# Autodesk Inventor assembly: X_Carriage_V2_1
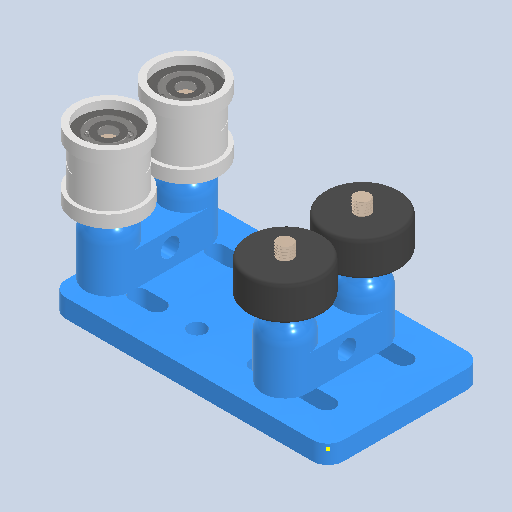
[picture p0: Inventor's stored thumbnail of the model, 512x512]
Saved by Autodesk Inventor 2022 (Build 260153000, 153)
## iProperties
Created: 2021-06-13
Part Number: X_Carriage_V2_1
Document SubType Name: Assembly
Designer: Jorian Brusind
Author: Jorian Brusind
## Documents named in this file (8)
- C:\Users\Jorian Brusind\Documents\GitHub\HyperRail\Inventor Files\X_Carriage_V2_1.iam
- C:\Users\Jorian Brusind\Documents\GitHub\HyperRail\Inventor Files\X_Carriage_Plate.ipt
- C:\Users\Jorian Brusind\Documents\GitHub\HyperRail\Inventor Files\11mm_BearingWheel.ipt
- C:\Users\Jorian Brusind\Documents\GitHub\HyperRail\Inventor Files\4mm_Roller_Spacer_extended.ipt
- C:\Users\Jorian Brusind\Documents\GitHub\HyperRail\Inventor Files\miniature-ball-bearings-metric-series-flanged-1.snapshot.1\F606ZZFlanged\F608 - 8 x 22 x 7.ipt
- C:\Users\Jorian Brusind\Documents\GitHub\PersonalProjects\HyperRail\Inventor Files\miniature-ball-bearings-metric-series-flanged-1.snapshot.1\F606ZZFlanged.ipt
- C:\Users\Jorian Brusind\Documents\GitHub\HyperRail\Inventor Files\685ZZFlanged_Adapter.ipt
- C:\Users\Jorian Brusind\Documents\GitHub\HyperRail\Inventor Files\Metric bolt\Bolt M5 45mm.ipt
## Components (17 placed, 6 different names)
1. X_Carriage_Plate:1 — Mate:51, Mate:53, Mate:65, Angle:1, Mate:66, Angle:2, Mate:98
2. 11mm_BearingWheel:1 — Flush:2, Mate:56, Mate:67
3. 11mm_BearingWheel:4 — Flush:2, Mate:57
4. 4mm_Roller_Spacer_extended:1 — Mate:53, Mate:56, Mate:57, Mate:66, Angle:2, Mate:67, Mate:96, Mate:97
5. 4mm_Roller_Spacer_extended:2 — Mate:51, Mate:65, Angle:1, Mate:76, Mate:77, Mate:78, Mate:79, Mate:94, Mate:95
6. F608 - 8 x 22 x 7:1 — Mate:78, Mate:89, Mate:91
7. F608 - 8 x 22 x 7:2 — Mate:76, Mate:90, Mate:92
8. F608 - 8 x 22 x 7:3 — Mate:79, Mate:84, Mate:85
9. F608 - 8 x 22 x 7:4 — Mate:77, Mate:86, Mate:87
10. 685ZZFlanged_Adapter:1 — Mate:86, Mate:87, Mate:88
11. 685ZZFlanged_Adapter:2 — Mate:84, Mate:85, Mate:88
12. 685ZZFlanged_Adapter:3 — Mate:89, Mate:91, Mate:93
13. 685ZZFlanged_Adapter:4 — Mate:90, Mate:92, Mate:93
14. Bolt M5 45mm:1 — Mate:94, Flush:3
15. Bolt M5 45mm:2 — Mate:96, Flush:5, Mate:98
16. Bolt M5 45mm:3 — Mate:97, Flush:4, Flush:5
17. Bolt M5 45mm:4 — Mate:95, Flush:3, Flush:4
## Relationships (34: Mate 28, Flush 4, Angle 2)
- Flush:2: 11mm_BearingWheel:1 ↔ 11mm_BearingWheel:4
- Mate:51: X_Carriage_Plate:1 ↔ 4mm_Roller_Spacer_extended:2
- Mate:53: X_Carriage_Plate:1 ↔ 4mm_Roller_Spacer_extended:1
- Mate:56: 11mm_BearingWheel:1 ↔ 4mm_Roller_Spacer_extended:1
- Mate:57: 11mm_BearingWheel:4 ↔ 4mm_Roller_Spacer_extended:1
- Mate:65 (-12.5 mm): X_Carriage_Plate:1 ↔ 4mm_Roller_Spacer_extended:2
- Angle:1 (0 deg): X_Carriage_Plate:1 ↔ 4mm_Roller_Spacer_extended:2
- Mate:66 (-12.5 mm): X_Carriage_Plate:1 ↔ 4mm_Roller_Spacer_extended:1
- Angle:2 (0 deg): X_Carriage_Plate:1 ↔ 4mm_Roller_Spacer_extended:1
- Mate:67: 11mm_BearingWheel:1 ↔ 4mm_Roller_Spacer_extended:1
- [Mate]: F608 - 8 x 22 x 7:1 ↔ F608 - 8 x 22 x 7:2
- [Mate]: F608 - 8 x 22 x 7:3 ↔ F608 - 8 x 22 x 7:4
- Mate:76: 4mm_Roller_Spacer_extended:2 ↔ F608 - 8 x 22 x 7:2
- Mate:77: 4mm_Roller_Spacer_extended:2 ↔ F608 - 8 x 22 x 7:4
- Mate:78: 4mm_Roller_Spacer_extended:2 ↔ F608 - 8 x 22 x 7:1
- Mate:79: 4mm_Roller_Spacer_extended:2 ↔ F608 - 8 x 22 x 7:3
- Mate:84: F608 - 8 x 22 x 7:3 ↔ 685ZZFlanged_Adapter:2
- Mate:85: F608 - 8 x 22 x 7:3 ↔ 685ZZFlanged_Adapter:2
- Mate:86: F608 - 8 x 22 x 7:4 ↔ 685ZZFlanged_Adapter:1
- Mate:87: F608 - 8 x 22 x 7:4 ↔ 685ZZFlanged_Adapter:1
- Mate:88: 685ZZFlanged_Adapter:1 ↔ 685ZZFlanged_Adapter:2
- Mate:89: F608 - 8 x 22 x 7:1 ↔ 685ZZFlanged_Adapter:3
- Mate:90: F608 - 8 x 22 x 7:2 ↔ 685ZZFlanged_Adapter:4
- Mate:91: F608 - 8 x 22 x 7:1 ↔ 685ZZFlanged_Adapter:3
- Mate:92: F608 - 8 x 22 x 7:2 ↔ 685ZZFlanged_Adapter:4
- Mate:93: 685ZZFlanged_Adapter:3 ↔ 685ZZFlanged_Adapter:4
- Mate:94: 4mm_Roller_Spacer_extended:2 ↔ Bolt M5 45mm:1
- Mate:95: 4mm_Roller_Spacer_extended:2 ↔ Bolt M5 45mm:4
- Mate:96: 4mm_Roller_Spacer_extended:1 ↔ Bolt M5 45mm:2
- Mate:97: 4mm_Roller_Spacer_extended:1 ↔ Bolt M5 45mm:3
- Flush:3: Bolt M5 45mm:1 ↔ Bolt M5 45mm:4
- Flush:4: Bolt M5 45mm:3 ↔ Bolt M5 45mm:4
- Flush:5: Bolt M5 45mm:2 ↔ Bolt M5 45mm:3
- Mate:98: X_Carriage_Plate:1 ↔ Bolt M5 45mm:2
## Named parameters: d136_d94 = 0 mm, d129_d136_d94 = 0 mm
